# Autodesk Inventor assembly: ABD_Version_0.1_leftleg
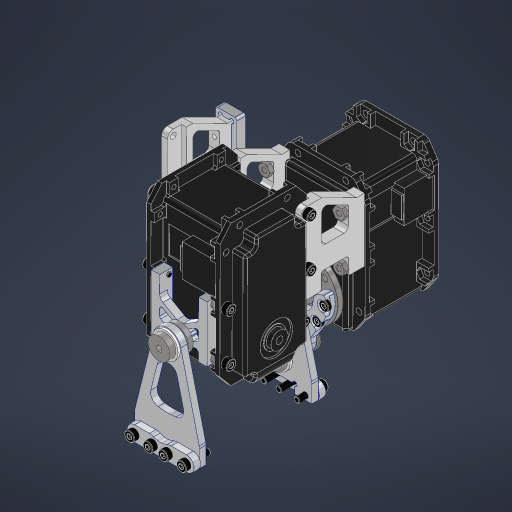
[picture p0: Inventor's stored thumbnail of the model, 512x512]
Saved by Autodesk Inventor 2024.3 (Build 283343000, 343)
## iProperties
Created: 2024-01-23
Part Number: ABD_Version_0.1_leftleg
Document SubType Name: Assembly
Designer: ASUS
Mass: 357.136 g
Surface Area: 604.848 cm^2
Volume: 181.423 cm^3
Density: 1.96853 g/cm^3
Author: ASUS
## Documents named in this file (19)
- C:\Users\ASUS\Desktop\Anti_Backlash_Structure_OP\v4_Frame_2025\ABD_V4_Left_OP.iam
- C:\Users\ASUS\Desktop\Anti_Backlash_Structure_OP\v4_Frame_2025\ABD_MX_64_Roll_Fixation_Set.iam
- C:\Users\ASUS\Desktop\Anti_Backlash_Structure_OP\v4_Frame_2025\Roll_Fixation_Frame_Back.ipt
- C:\Users\ASUS\Desktop\Anti_Backlash_Structure_OP\v4_Frame_2025\hip joint fix washer.ipt
- C:\Users\ASUS\Desktop\Anti_Backlash_Structure_OP\MISUMI\hip_joint_fix_washer_10mm_Set.iam
- C:\Users\ASUS\Desktop\Anti_Backlash_Structure_OP\v4_Frame_2025\Front_Frame_Fixer_v2.iam
- C:\Users\ASUS\Desktop\Anti_Backlash_Structure_OP\ROBOTIS(Inventor 2024 ver.)\DXL\MX-64T.ipt
- C:\Users\ASUS\Desktop\Anti_Backlash_Structure_OP\v4_Frame_2025\Dynamixel Vertical fixation.ipt
- C:\Users\ASUS\Desktop\Anti_Backlash_Structure_OP\v4_Frame_2025\Dynamixel Vertical fixation_MIR.ipt
- C:\Users\ASUS\Desktop\Anti_Backlash_Structure_OP\MISUMI\SLBNR2_5.ipt
- C:\Users\ASUS\Desktop\Anti_Backlash_Structure_OP\MISUMI\Roll_Fixation_Frame_8mm_Set.iam
- C:\Users\ASUS\Desktop\Anti_Backlash_Structure_OP\MISUMI\Roll_Fixation_Frame_8mm_Set_Backside.iam
- C:\Users\ASUS\Desktop\Anti_Backlash_Structure_OP\v4_Frame_2025\Roll_Fixation_Frame.ipt
- C:\Users\ASUS\Desktop\Anti_Backlash_Structure_OP\V2_Frame(2025)\Slider_crank_horn_v2_2025.ipt
- C:\Users\ASUS\Desktop\Anti_Backlash_Structure_OP\ROBOTIS(Inventor 2024 ver.)\HORN\64-106Horn.ipt
- C:\Users\ASUS\Desktop\Anti_Backlash_Structure_OP\MISUMI\CSHBTT-SUS-M2.5-4.ipt
- C:\Users\ASUS\Desktop\Anti_Backlash_Structure_OP\MISUMI\CSH-STN-M3-10_203.ipt
- C:\Users\ASUS\Desktop\Anti_Backlash_Structure_OP\v4_Frame_2025\ALI\Crank_Fixation.iam
- C:\Users\ASUS\Desktop\Anti_Backlash_Structure_OP\v4_Frame_2025\Zig.ipt
## Components (28 placed, 18 different names)
1. hip joint fix washer:1 — 메이트:50
2. hip joint fix washer:2 — 삽입:47, 메이트:29
3. hip_joint_fix_washer_10mm_Set:1 [sub-assembly] — 메이트:49, 메이트:50
4. hip_joint_fix_washer_10mm_Set:2 [sub-assembly] — 메이트:29, 메이트:43
5. Front_Frame_Fixer_v2:1 [sub-assembly] — 삽입:46, 삽입:74
6. ABD_MX_64_Roll_Fixation_Set:2 [sub-assembly] — 각도:3, 플러쉬:1, 삽입:46, 삽입:71, 메이트:45, 삽입:72, 메이트:46, 삽입:78
7. MX-64T:1 — 각도:3, 플러쉬:1, 메이트:36, 메이트:51, 메이트:52, 메이트:54, 플러쉬:2, 메이트:60, 메이트:61
8. Roll_Fixation_Frame_Back:3 — 삽입:47, 메이트:43, 삽입:79, 메이트:55, 메이트:56
9. Dynamixel Vertical fixation:2 — 메이트:47, 메이트:48, 메이트:51, 메이트:52, 플러쉬:3, 플러쉬:4
10. Dynamixel Vertical fixation_MIR:2 — 메이트:36, 메이트:58, 메이트:59, 메이트:60
11. SLBNR2_5:5
12. SLBNR2_5:6
13. SLBNR2_5:7
14. SLBNR2_5:8
15. Roll_Fixation_Frame_8mm_Set:1 [sub-assembly] — 삽입:71, 메이트:45
16. Roll_Fixation_Frame_8mm_Set_Backside:1 [sub-assembly] — 삽입:72, 메이트:46, 메이트:47, 메이트:48, 메이트:58, 메이트:59
17. Roll_Fixation_Frame:1 — 삽입:74, 메이트:49
18. Front_Frame_Fixer_v2:2 [sub-assembly] — 삽입:78, 삽입:79
19. 64-106Horn:1 — 삽입:81, 메이트:53, 메이트:54, 플러쉬:2, 삽입:86
20. Slider_crank_horn_v2_2025:1 — 삽입:81, 메이트:53, 삽입:82, 삽입:83, 삽입:84, 삽입:85, 메이트:57
21. CSHBTT-SUS-M2.5-4:2 — 삽입:84
22. CSHBTT-SUS-M2.5-4:3 — 삽입:85
23. CSHBTT-SUS-M2.5-4:4 — 삽입:83
24. CSHBTT-SUS-M2.5-4:5 — 삽입:82
25. CSH-STN-M3-10_203:1 — 삽입:86
26. Crank_Fixation:1 [sub-assembly] — 메이트:55, 메이트:56, 메이트:57
27. Dynamixel Vertical fixation:3 — 플러쉬:3, 메이트:61, 플러쉬:4, 삽입:87, 메이트:62
28. Zig:1 — 삽입:87, 메이트:62
## Relationships (52: Mate 25, Insert 20, Flush 4, Angle 3)
- [Insert]: hip joint fix washer:1 ↔ hip_joint_fix_washer_10mm_Set:1
- [Mate]: hip joint fix washer:1 ↔ hip_joint_fix_washer_10mm_Set:1
- [Insert]: hip joint fix washer:2 ↔ hip_joint_fix_washer_10mm_Set:2
- [Mate]: hip joint fix washer:2 ↔ hip_joint_fix_washer_10mm_Set:2
- [Mate]: hip_joint_fix_washer_10mm_Set:1 ↔ hip_joint_fix_washer_10mm_Set:2
- [Mate]: hip_joint_fix_washer_10mm_Set:1 ↔ hip_joint_fix_washer_10mm_Set:2
- 각도:3 [Angle] (0 deg): ABD_MX_64_Roll_Fixation_Set:2 ↔ MX-64T:1
- 플러쉬:1 [Flush] (-3.1 mm): ABD_MX_64_Roll_Fixation_Set:2 ↔ MX-64T:1
- 삽입:46 [Insert]: Front_Frame_Fixer_v2:1 ↔ ABD_MX_64_Roll_Fixation_Set:2
- 삽입:47 [Insert]: hip joint fix washer:2 ↔ Roll_Fixation_Frame_Back:3
- 메이트:29 [Mate]: hip joint fix washer:2 ↔ hip_joint_fix_washer_10mm_Set:2
- [Insert]: Dynamixel Vertical fixation:2 ↔ SLBNR2_5:5
- [Insert]: Dynamixel Vertical fixation:2 ↔ SLBNR2_5:6
- [Insert]: Dynamixel Vertical fixation_MIR:2 ↔ SLBNR2_5:8
- [Insert]: Dynamixel Vertical fixation_MIR:2 ↔ SLBNR2_5:7
- [Angle] (0 deg): Dynamixel Vertical fixation_MIR:2 ↔ SLBNR2_5:7
- [Angle] (0 deg): Dynamixel Vertical fixation_MIR:2 ↔ SLBNR2_5:8
- 메이트:36 [Mate]: MX-64T:1 ↔ Dynamixel Vertical fixation_MIR:2
- 메이트:43 [Mate]: hip_joint_fix_washer_10mm_Set:2 ↔ Roll_Fixation_Frame_Back:3
- 삽입:71 [Insert]: ABD_MX_64_Roll_Fixation_Set:2 ↔ Roll_Fixation_Frame_8mm_Set:1
- 메이트:45 [Mate]: ABD_MX_64_Roll_Fixation_Set:2 ↔ Roll_Fixation_Frame_8mm_Set:1
- 삽입:72 [Insert]: ABD_MX_64_Roll_Fixation_Set:2 ↔ Roll_Fixation_Frame_8mm_Set_Backside:1
- 메이트:46 [Mate]: ABD_MX_64_Roll_Fixation_Set:2 ↔ Roll_Fixation_Frame_8mm_Set_Backside:1
- 메이트:47 [Mate]: Dynamixel Vertical fixation:2 ↔ Roll_Fixation_Frame_8mm_Set_Backside:1
- 메이트:48 [Mate]: Dynamixel Vertical fixation:2 ↔ Roll_Fixation_Frame_8mm_Set_Backside:1
- 삽입:74 [Insert]: Front_Frame_Fixer_v2:1 ↔ Roll_Fixation_Frame:1
- 메이트:49 [Mate]: hip_joint_fix_washer_10mm_Set:1 ↔ Roll_Fixation_Frame:1
- 메이트:50 [Mate]: hip joint fix washer:1 ↔ hip_joint_fix_washer_10mm_Set:1
- 삽입:78 [Insert]: ABD_MX_64_Roll_Fixation_Set:2 ↔ Front_Frame_Fixer_v2:2
- 삽입:79 [Insert]: Roll_Fixation_Frame_Back:3 ↔ Front_Frame_Fixer_v2:2
- 메이트:51 [Mate]: MX-64T:1 ↔ Dynamixel Vertical fixation:2
- 메이트:52 [Mate]: MX-64T:1 ↔ Dynamixel Vertical fixation:2
- 삽입:81 [Insert]: 64-106Horn:1 ↔ Slider_crank_horn_v2_2025:1
- 메이트:53 [Mate]: 64-106Horn:1 ↔ Slider_crank_horn_v2_2025:1
- 삽입:82 [Insert]: Slider_crank_horn_v2_2025:1 ↔ CSHBTT-SUS-M2.5-4:5
- 삽입:83 [Insert]: Slider_crank_horn_v2_2025:1 ↔ CSHBTT-SUS-M2.5-4:4
- 삽입:84 [Insert]: Slider_crank_horn_v2_2025:1 ↔ CSHBTT-SUS-M2.5-4:2
- 삽입:85 [Insert]: Slider_crank_horn_v2_2025:1 ↔ CSHBTT-SUS-M2.5-4:3
- 메이트:54 [Mate]: MX-64T:1 ↔ 64-106Horn:1
- 플러쉬:2 [Flush] (-3 mm): MX-64T:1 ↔ 64-106Horn:1
- 삽입:86 [Insert]: 64-106Horn:1 ↔ CSH-STN-M3-10_203:1
- 메이트:55 [Mate]: Roll_Fixation_Frame_Back:3 ↔ Crank_Fixation:1
- 메이트:56 [Mate]: Roll_Fixation_Frame_Back:3 ↔ Crank_Fixation:1
- 메이트:57 [Mate]: Slider_crank_horn_v2_2025:1 ↔ Crank_Fixation:1
- 메이트:58 [Mate]: Dynamixel Vertical fixation_MIR:2 ↔ Roll_Fixation_Frame_8mm_Set_Backside:1
- 메이트:59 [Mate]: Dynamixel Vertical fixation_MIR:2 ↔ Roll_Fixation_Frame_8mm_Set_Backside:1
- 메이트:60 [Mate]: MX-64T:1 ↔ Dynamixel Vertical fixation_MIR:2
- 플러쉬:3 [Flush] (25 mm): Dynamixel Vertical fixation:2 ↔ Dynamixel Vertical fixation:3
- 메이트:61 [Mate]: MX-64T:1 ↔ Dynamixel Vertical fixation:3
- 플러쉬:4 [Flush]: Dynamixel Vertical fixation:2 ↔ Dynamixel Vertical fixation:3
- 삽입:87 [Insert]: Dynamixel Vertical fixation:3 ↔ Zig:1
- 메이트:62 [Mate]: Dynamixel Vertical fixation:3 ↔ Zig:1
## Named parameters: d1061_d1053 = 0 mm, d1062_d1054 = 0 mm, d1063_d1055 = 0 mm, d1064_d1056 = 0 mm, d1065_d1057 = 0 deg, d1066_d1058 = 0 deg
